# Autodesk Inventor assembly: ResistojetPrototype
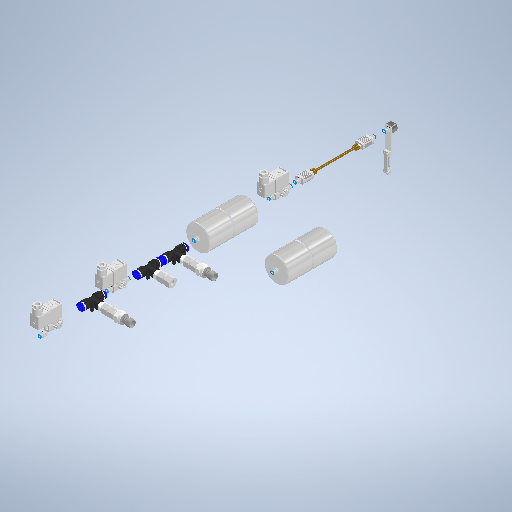
[picture p0: Inventor's stored thumbnail of the model, 512x512]
Saved by Autodesk Inventor 2025.2 (Build 292293000, 293)
## iProperties
Created: 2026-06-11
Part Number: ResistojetPrototype
Document SubType Name: Assembly
Designer: Simon
Author: Simon
## Documents named in this file (16)
- C:\Users\Simon\Projects\MEng Electronics\Development of a Resistojet Thruster\3) Hardware\Resistojet Design\ThrusterV3\ResistojetPrototype.iam
- C:\Users\Simon\Projects\MEng Electronics\Development of a Resistojet Thruster\3) Hardware\Resistojet Design\ThrusterV3\Mechanical Drawings\Heater.ipt
- C:\Users\Simon\Projects\MEng Electronics\Development of a Resistojet Thruster\3) Hardware\Resistojet Design\ThrusterV3\PressureSensor.ipt
- C:\Users\Simon\Projects\MEng Electronics\Development of a Resistojet Thruster\3) Hardware\Resistojet Design\ThrusterV3\Festo_Pneumatic_Coupling_PC4-M10.ipt
- C:\Users\Simon\Projects\MEng Electronics\Development of a Resistojet Thruster\3) Hardware\Resistojet Design\ThrusterV3\Creality Heatsink v1.2.ipt
- C:\Users\Simon\Projects\MEng Electronics\Development of a Resistojet Thruster\3) Hardware\Resistojet Design\ThrusterV3\Heatbreak CR30.ipt
- C:\Users\Simon\Projects\MEng Electronics\Development of a Resistojet Thruster\3) Hardware\Resistojet Design\ThrusterV3\NozzleConnector.ipt
- C:\Users\Simon\Projects\MEng Electronics\Development of a Resistojet Thruster\3) Hardware\Resistojet Design\ThrusterV3\0.4 nozzle.ipt
- C:\Users\Simon\Projects\MEng Electronics\Development of a Resistojet Thruster\3) Hardware\Resistojet Design\ThrusterV3\100g_load_cell.ipt
- C:\Users\Simon\Projects\MEng Electronics\Development of a Resistojet Thruster\3) Hardware\Resistojet Design\ThrusterV3\Loadcell_lever.ipt
- C:\Users\Simon\Projects\MEng Electronics\Development of a Resistojet Thruster\3) Hardware\Resistojet Design\ThrusterV3\ASCO Solenoid Valve\solenoid_valve_scg256a004nvms_4.iam
- C:\Users\Simon\Projects\MEng Electronics\Development of a Resistojet Thruster\3) Hardware\Resistojet Design\ThrusterV3\TeePushFit\131.014-10.iam
- C:\Users\Simon\Projects\MEng Electronics\Development of a Resistojet Thruster\3) Hardware\Resistojet Design\ThrusterV3\103hss1_4.ipt
- C:\Users\Simon\Projects\MEng Electronics\Development of a Resistojet Thruster\3) Hardware\Resistojet Design\ThrusterV3\119hss1_4x1_8.ipt
- C:\Users\Simon\Projects\MEng Electronics\Development of a Resistojet Thruster\3) Hardware\Resistojet Design\ThrusterV3\Mechanical Drawings\WeldedPlenumAssembly.iam
- C:\Users\Simon\Projects\MEng Electronics\Development of a Resistojet Thruster\3) Hardware\Resistojet Design\ThrusterV3\Mechanical Drawings\WeldedTankAssembly.iam
## Components (33 placed, 15 different names)
1. Heater:1 — Mate:35, Mate:36, Mate:43, Mate:44
2. PressureSensor:2 — Mate:61, Mate:63
3. Festo_Pneumatic_Coupling_PC4-M10:1 — Mate:54, Mate:56
4. Festo_Pneumatic_Coupling_PC4-M10:2 — Mate:47, Mate:48, Mate:49
5. Festo_Pneumatic_Coupling_PC4-M10:3 — Mate:55, Mate:57
6. Festo_Pneumatic_Coupling_PC4-M10:4 — Mate:37, Mate:38
7. Festo_Pneumatic_Coupling_PC4-M10:5 — Mate:74, Mate:75
8. Festo_Pneumatic_Coupling_PC4-M10:6
9. Creality Heatsink v1.2:1 — Mate:33, Mate:34, Mate:37, Mate:38
10. Heatbreak CR30:1 — Mate:33, Mate:34, Mate:35, Mate:36
11. Festo_Pneumatic_Coupling_PC4-M10:7
12. Creality Heatsink v1.2:2
13. Heatbreak CR30:2 — Mate:43, Mate:44
14. NozzleConnector:1 — Mate:45, Mate:46, Mate:47, Mate:50
15. 0.4 nozzle:1 — Mate:45, Mate:46
16. 100g_load_cell:1 — Mate:51, Mate:52, Mate:53
17. Loadcell_lever:1 — Mate:48, Mate:49, Mate:50, Mate:51, Mate:52, Mate:53
18. solenoid_valve_scg256a004nvms_4:1 [sub-assembly] — Mate:58, Mate:59, Mate:68, Mate:69
19. solenoid_valve_scg256a004nvms_4:2 [sub-assembly] — Mate:54, Mate:55, Mate:56, Mate:57
20. solenoid_valve_scg256a004nvms_4:3 [sub-assembly]
21. Festo_Pneumatic_Coupling_PC4-M10:8 — Mate:59, Mate:68
22. Festo_Pneumatic_Coupling_PC4-M10:9 — Mate:58, Mate:69
23. 131.014-10:1 [sub-assembly] — Mate:60, Mate:62
24. 103hss1_4:1 — Mate:60, Mate:61, Mate:62, Mate:63
25. PressureSensor:4
26. 131.014-10:2 [sub-assembly]
27. 103hss1_4:2
28. 131.014-10:3 [sub-assembly] — Mate:70, Mate:71
29. 119hss1_4x1_8:1 — Mate:70, Mate:71
30. Festo_Pneumatic_Coupling_PC4-M10:10 — Mate:73, Mate:77
31. Festo_Pneumatic_Coupling_PC4-M10:11 — Mate:72, Mate:76
32. WeldedPlenumAssembly:1 [sub-assembly] — Mate:72, Mate:73, Mate:76, Mate:77
33. WeldedTankAssembly:1 [sub-assembly] — Mate:74, Mate:75
## Relationships (45: Mate 45)
- Mate:33: Creality Heatsink v1.2:1 ↔ Heatbreak CR30:1
- Mate:34: Creality Heatsink v1.2:1 ↔ Heatbreak CR30:1
- Mate:35: Heater:1 ↔ Heatbreak CR30:1
- Mate:36: Heater:1 ↔ Heatbreak CR30:1
- Mate:37: Festo_Pneumatic_Coupling_PC4-M10:4 ↔ Creality Heatsink v1.2:1
- Mate:38: Festo_Pneumatic_Coupling_PC4-M10:4 ↔ Creality Heatsink v1.2:1
- [Mate]: Creality Heatsink v1.2:2 ↔ Heatbreak CR30:2
- [Mate]: Creality Heatsink v1.2:2 ↔ Heatbreak CR30:2
- [Mate]: Festo_Pneumatic_Coupling_PC4-M10:7 ↔ Creality Heatsink v1.2:2
- [Mate]: Festo_Pneumatic_Coupling_PC4-M10:7 ↔ Creality Heatsink v1.2:2
- Mate:43: Heater:1 ↔ Heatbreak CR30:2
- Mate:44: Heater:1 ↔ Heatbreak CR30:2
- Mate:45: NozzleConnector:1 ↔ 0.4 nozzle:1
- Mate:46: NozzleConnector:1 ↔ 0.4 nozzle:1
- Mate:47: Festo_Pneumatic_Coupling_PC4-M10:2 ↔ NozzleConnector:1
- Mate:48: Festo_Pneumatic_Coupling_PC4-M10:2 ↔ Loadcell_lever:1
- Mate:49: Festo_Pneumatic_Coupling_PC4-M10:2 ↔ Loadcell_lever:1
- Mate:50: NozzleConnector:1 ↔ Loadcell_lever:1
- Mate:51: 100g_load_cell:1 ↔ Loadcell_lever:1
- Mate:52: 100g_load_cell:1 ↔ Loadcell_lever:1
- Mate:53: 100g_load_cell:1 ↔ Loadcell_lever:1
- Mate:54: Festo_Pneumatic_Coupling_PC4-M10:1 ↔ solenoid_valve_scg256a004nvms_4:2
- Mate:55: Festo_Pneumatic_Coupling_PC4-M10:3 ↔ solenoid_valve_scg256a004nvms_4:2
- Mate:56: Festo_Pneumatic_Coupling_PC4-M10:1 ↔ solenoid_valve_scg256a004nvms_4:2
- Mate:57: Festo_Pneumatic_Coupling_PC4-M10:3 ↔ solenoid_valve_scg256a004nvms_4:2
- Mate:58: solenoid_valve_scg256a004nvms_4:1 ↔ Festo_Pneumatic_Coupling_PC4-M10:9
- Mate:59: solenoid_valve_scg256a004nvms_4:1 ↔ Festo_Pneumatic_Coupling_PC4-M10:8
- Mate:60: 131.014-10:1 ↔ 103hss1_4:1
- Mate:61: PressureSensor:2 ↔ 103hss1_4:1
- Mate:62: 131.014-10:1 ↔ 103hss1_4:1
- Mate:63: PressureSensor:2 ↔ 103hss1_4:1
- [Mate]: 131.014-10:2 ↔ 103hss1_4:2
- [Mate]: PressureSensor:4 ↔ 103hss1_4:2
- [Mate]: 131.014-10:2 ↔ 103hss1_4:2
- [Mate]: PressureSensor:4 ↔ 103hss1_4:2
- Mate:68: solenoid_valve_scg256a004nvms_4:1 ↔ Festo_Pneumatic_Coupling_PC4-M10:8
- Mate:69: solenoid_valve_scg256a004nvms_4:1 ↔ Festo_Pneumatic_Coupling_PC4-M10:9
- Mate:70: 131.014-10:3 ↔ 119hss1_4x1_8:1
- Mate:71: 131.014-10:3 ↔ 119hss1_4x1_8:1
- Mate:72: Festo_Pneumatic_Coupling_PC4-M10:11 ↔ WeldedPlenumAssembly:1
- Mate:73: Festo_Pneumatic_Coupling_PC4-M10:10 ↔ WeldedPlenumAssembly:1
- Mate:74: Festo_Pneumatic_Coupling_PC4-M10:5 ↔ WeldedTankAssembly:1
- Mate:75: Festo_Pneumatic_Coupling_PC4-M10:5 ↔ WeldedTankAssembly:1
- Mate:76: Festo_Pneumatic_Coupling_PC4-M10:11 ↔ WeldedPlenumAssembly:1
- Mate:77: Festo_Pneumatic_Coupling_PC4-M10:10 ↔ WeldedPlenumAssembly:1
## Named parameters: d43_d37 = 0 mm, d44_d38 = 0 mm, d45_d41 = 0 mm, d46_d42 = 0 mm, d69_d65 = 0 mm, d70_d66 = 0 mm, d71_d67 = 0 mm, d72_d68 = 0 mm
